# Autodesk Inventor assembly: middleMale
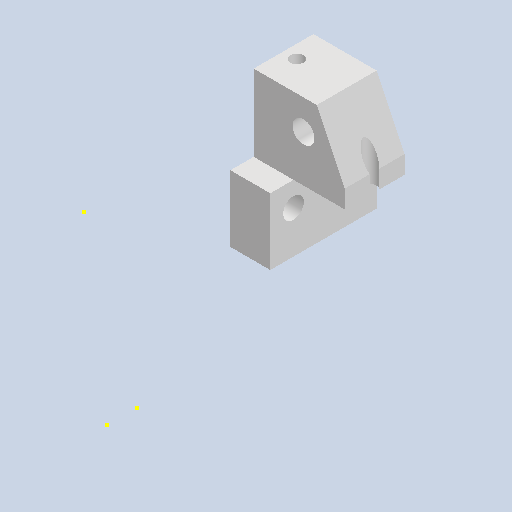
[picture p0: Inventor's stored thumbnail of the model, 512x512]
Saved by Autodesk Inventor 2024 (Build 280153000, 153)
## iProperties
Created: 2024-06-10
Part Number: middleMale
Document SubType Name: Assembly
Designer: omiye
Author: omiye
## Documents named in this file (3)
- C:\Projects\roboticHand\fingerModels\mfP2.iam
- C:\Projects\roboticHand\fingerModels\mfP1.ipt
- C:\Projects\roboticHand\fingerModels\normMale.ipt
## Components (2 placed, 2 different names)
1. middleFingerMale:1 — Mate:1, Mate:2
2. normMale:1 — Mate:1, Mate:2
## Relationships (2: Mate 2)
- Mate:1: middleFingerMale:1 ↔ normMale:1
- Mate:2: middleFingerMale:1 ↔ normMale:1
